# Autodesk Inventor assembly: FarmBot
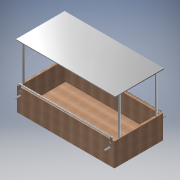
[picture p0: Inventor's stored thumbnail of the model, 180x180]
Saved by Autodesk Inventor 2017 (Build 210142000, 142)
## iProperties
Created: 2016-12-12
Part Number: FarmBot
Document SubType Name: Assembly
Designer: umr
Author: umr
## Documents named in this file (6)
- D:\SeniorProject\Models2\FarmBot.iam
- D:\SeniorProject\Models2\BedAssembly\BedAseembly.iam
- D:\SeniorProject\Models2\Gantry\GantryDown.iam
- D:\SeniorProject\Models2\Gantry\GantryUp.iam
- D:\SeniorProject\Models2\Case\Case.iam
- D:\SeniorProject\Models2\LED Structure\LED Structure Assembly.iam
## Components (5 placed, 5 different names)
1. BedAseembly:2 [sub-assembly] — Mate:9, Tangent:2, Mate:10, Mate:11, Mate:12, Mate:13, Flush:2, Mate:14, Mate:15, Mate:16
2. GantryDown:1 [sub-assembly] — Mate:9, Tangent:2, Flush:2, Mate:17
3. Case:1 [sub-assembly] — Mate:10, Mate:11, Mate:12, Mate:13
4. LED Structure Assembly:1 [sub-assembly] — Mate:14, Mate:15, Mate:16
5. GantryUp:1 [sub-assembly] — Mate:17
## Relationships (11: Mate 9, Tangent 1, Flush 1)
- Mate:9: BedAseembly:2 ↔ GantryDown:1
- Tangent:2: BedAseembly:2 ↔ GantryDown:1
- Mate:10: BedAseembly:2 ↔ Case:1
- Mate:11: BedAseembly:2 ↔ Case:1
- Mate:12: BedAseembly:2 ↔ Case:1
- Mate:13: BedAseembly:2 ↔ Case:1
- Flush:2 (200 mm): BedAseembly:2 ↔ GantryDown:1
- Mate:14: BedAseembly:2 ↔ LED Structure Assembly:1
- Mate:15: BedAseembly:2 ↔ LED Structure Assembly:1
- Mate:16: BedAseembly:2 ↔ LED Structure Assembly:1
- Mate:17: GantryDown:1 ↔ GantryUp:1
